# Autodesk Inventor assembly: rotation base断面図_
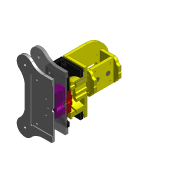
[picture p0: Inventor's stored thumbnail of the model, 180x180]
Saved by Autodesk Inventor 2013 (Build 170138000, 138)
## iProperties
Created: 2012-10-15
Part Number: rotation base断面図_
Document SubType Name: Assembly
Designer: JohnHenry
Mass: 215.328 g
Surface Area: 1206.82 cm^2
Volume: 215.328 cm^3
Density: 1 g/cm^3
Author: JohnHenry
## Documents named in this file (15)
- C:\Users\victor\Desktop\Documents\Inventor\walkPivot\rotation base断面図_.iam
- C:\Users\victor\Desktop\Documents\Inventor\walkPivot\JointB0.ipt
- C:\Users\victor\Desktop\Documents\Inventor\walkPivot\JointB1.ipt
- C:\Users\victor\Desktop\Documents\Inventor\walkPivot\80F-5020.ipt
- C:\Users\victor\Desktop\Documents\Inventor\walkPivot\JointB2.ipt
- C:\Users\victor\Desktop\Documents\Inventor\walkPivot\JointA2.ipt
- C:\Users\victor\Desktop\Documents\Inventor\walkPivot\JointA1.ipt
- C:\Users\victor\Desktop\Documents\Inventor\walkPivot\JointA0.ipt
- C:\Users\victor\Desktop\Documents\Inventor\walkPivot\JointA3.ipt
- C:\Users\victor\Desktop\Documents\Inventor\walkPivot\walkingCDGA\SLIPRING_SRG-1-6G.iam
- C:\Users\victor\Desktop\Documents\Inventor\walkPivot\ベアリング(仮).ipt
- C:\Users\victor\Desktop\Documents\Inventor\walkPivot\JointB0_.ipt
- C:\Users\victor\Desktop\Documents\Inventor\walkPivot\JointC0_.ipt
- C:\Users\victor\Desktop\Documents\Inventor\walkPivot\HEDS-5500_A.ipt
- C:\Users\victor\Desktop\Documents\Inventor\walkPivot\HEDS-5500_B.ipt
## Components (23 placed, 14 different names)
1. JointB1:1 — メイト:1, フラッシュ:7, メイト:2, フラッシュ:19, フラッシュ:21, フラッシュ:22
2. JointB1:2 — フラッシュ:18, フラッシュ:20, フラッシュ:23, メイト:43, メイト:44, フラッシュ:35
3. 80F-5020:1 — 挿入:2, 挿入:5, 挿入:43
4. JointB2:1 — メイト:1, フラッシュ:7, メイト:2
5. JointA2:1 — 挿入:2, フラッシュ:8, フラッシュ:9, フラッシュ:10, フラッシュ:12, フラッシュ:13, フラッシュ:14, フラッシュ:15, 角度:7
6. JointA1:1 — フラッシュ:8, フラッシュ:9, 挿入:3, 挿入:4, フラッシュ:11, フラッシュ:16, フラッシュ:17
7. JointA0:1 — 挿入:3, 挿入:4, メイト:6, 挿入:42, 挿入:48, 挿入:49, 挿入:50, 挿入:51, メイト:53, メイト:54, メイト:55
8. JointA3:1 — フラッシュ:10, フラッシュ:11, フラッシュ:14, フラッシュ:17
9. JointA3:2 — フラッシュ:12, フラッシュ:13, フラッシュ:15, フラッシュ:16
10. JointB0:1 — 挿入:5, フラッシュ:18, フラッシュ:19, フラッシュ:20, フラッシュ:21, フラッシュ:22, フラッシュ:23, 角度:7, メイト:42
11. SLIPRING_SRG-1-6G:1 [sub-assembly] — メイト:6, 挿入:50, 挿入:51
12. ベアリング(仮):1 — 挿入:46
13. ベアリング(仮):2 — 挿入:45
14. ベアリング(仮):3 — 挿入:44
15. ベアリング(仮):4 — 挿入:47
16. ベアリング(仮):13 — 挿入:42
17. JointB0_:1 — メイト:42, 挿入:43
18. JointB2:2 — メイト:43, メイト:44, フラッシュ:35, メイト:45, フラッシュ:36, メイト:47, フラッシュ:37, メイト:49, メイト:50
19. JointC0_:1 — メイト:47, フラッシュ:37, メイト:50, 挿入:45, 挿入:46
20. JointC0_:2 — メイト:45, フラッシュ:36, メイト:49, 挿入:44, 挿入:47
21. HEDS-5500_A:1 — 挿入:48, 挿入:49, メイト:51, フラッシュ:38, メイト:52
22. HEDS-5500_B:1 — メイト:51, フラッシュ:38, メイト:52
23. JointA0:2 — メイト:53, メイト:54, メイト:55
## Relationships (51: Flush 21, Mate 15, Insert 14, Angle 1)
- メイト:1 [Mate] (0.1 mm): JointB1:1 ↔ JointB2:1
- フラッシュ:7 [Flush]: JointB1:1 ↔ JointB2:1
- メイト:2 [Mate]: JointB1:1 ↔ JointB2:1
- 挿入:2 [Insert]: 80F-5020:1 ↔ JointA2:1
- フラッシュ:8 [Flush]: JointA2:1 ↔ JointA1:1
- フラッシュ:9 [Flush]: JointA2:1 ↔ JointA1:1
- 挿入:3 [Insert]: JointA1:1 ↔ JointA0:1
- 挿入:4 [Insert]: JointA1:1 ↔ JointA0:1
- フラッシュ:10 [Flush]: JointA2:1 ↔ JointA3:1
- フラッシュ:11 [Flush]: JointA1:1 ↔ JointA3:1
- フラッシュ:12 [Flush]: JointA2:1 ↔ JointA3:2
- フラッシュ:13 [Flush]: JointA2:1 ↔ JointA3:2
- フラッシュ:14 [Flush]: JointA2:1 ↔ JointA3:1
- フラッシュ:15 [Flush]: JointA2:1 ↔ JointA3:2
- フラッシュ:16 [Flush]: JointA1:1 ↔ JointA3:2
- フラッシュ:17 [Flush]: JointA1:1 ↔ JointA3:1
- 挿入:5 [Insert]: 80F-5020:1 ↔ JointB0:1
- フラッシュ:18 [Flush]: JointB1:2 ↔ JointB0:1
- フラッシュ:19 [Flush]: JointB1:1 ↔ JointB0:1
- フラッシュ:20 [Flush]: JointB1:2 ↔ JointB0:1
- フラッシュ:21 [Flush]: JointB1:1 ↔ JointB0:1
- フラッシュ:22 [Flush]: JointB1:1 ↔ JointB0:1
- フラッシュ:23 [Flush]: JointB1:2 ↔ JointB0:1
- メイト:6 [Mate]: JointA0:1 ↔ SLIPRING_SRG-1-6G:1
- 角度:7 [Angle] (0 deg): JointA2:1 ↔ JointB0:1
- 挿入:42 [Insert] (0.5 mm): JointA0:1 ↔ ベアリング(仮):13
- メイト:42 [Mate]: JointB0:1 ↔ JointB0_:1
- 挿入:43 [Insert] (0.1 mm): 80F-5020:1 ↔ JointB0_:1
- メイト:43 [Mate] (0.1 mm): JointB1:2 ↔ JointB2:2
- メイト:44 [Mate]: JointB1:2 ↔ JointB2:2
- フラッシュ:35 [Flush]: JointB1:2 ↔ JointB2:2
- メイト:45 [Mate]: JointB2:2 ↔ JointC0_:2
- フラッシュ:36 [Flush]: JointB2:2 ↔ JointC0_:2
- メイト:47 [Mate]: JointB2:2 ↔ JointC0_:1
- フラッシュ:37 [Flush]: JointB2:2 ↔ JointC0_:1
- メイト:49 [Mate]: JointB2:2 ↔ JointC0_:2
- メイト:50 [Mate]: JointB2:2 ↔ JointC0_:1
- 挿入:44 [Insert]: ベアリング(仮):3 ↔ JointC0_:2
- 挿入:45 [Insert]: ベアリング(仮):2 ↔ JointC0_:1
- 挿入:46 [Insert]: ベアリング(仮):1 ↔ JointC0_:1
- 挿入:47 [Insert]: ベアリング(仮):4 ↔ JointC0_:2
- 挿入:48 [Insert]: JointA0:1 ↔ HEDS-5500_A:1
- 挿入:49 [Insert]: JointA0:1 ↔ HEDS-5500_A:1
- メイト:51 [Mate]: HEDS-5500_A:1 ↔ HEDS-5500_B:1
- フラッシュ:38 [Flush]: HEDS-5500_A:1 ↔ HEDS-5500_B:1
- メイト:52 [Mate]: HEDS-5500_A:1 ↔ HEDS-5500_B:1
- 挿入:50 [Insert]: JointA0:1 ↔ SLIPRING_SRG-1-6G:1
- 挿入:51 [Insert]: JointA0:1 ↔ SLIPRING_SRG-1-6G:1
- メイト:53 [Mate]: JointA0:1 ↔ JointA0:2
- メイト:54 [Mate] (20 mm): JointA0:1 ↔ JointA0:2
- メイト:55 [Mate]: JointA0:1 ↔ JointA0:2
